# Autodesk Inventor assembly: V2Leg
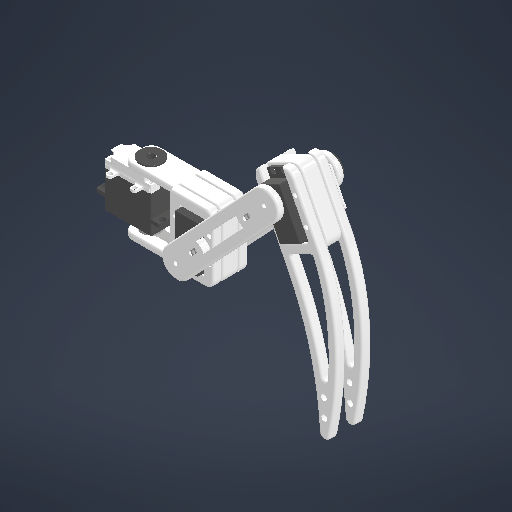
[picture p0: Inventor's stored thumbnail of the model, 512x512]
Saved by Autodesk Inventor 2026.2 (Build 302298010, 298A)
## iProperties
Created: 2026-02-21
Part Number: V2Leg
Document SubType Name: Assembly
Designer: Liam
Author: Liam
## Documents named in this file (12)
- C:\Users\Liam\OneDrive\Documents\Inventor\Hexapod\V2\V2Leg.iam
- C:\Users\Liam\OneDrive\Documents\Inventor\Hexapod\V2\TibiaRight.ipt
- C:\Users\Liam\OneDrive\Documents\Inventor\Hexapod\V2\ServoMount.ipt
- C:\Users\Liam\OneDrive\Documents\Inventor\Hexapod\V2\ServoAssembly.iam
- C:\Users\Liam\OneDrive\Documents\Inventor\Hexapod\V2\TibiaLeft.ipt
- C:\Users\Liam\OneDrive\Documents\Inventor\Hexapod\V2\FemurHornSide.ipt
- C:\Users\Liam\OneDrive\Documents\Inventor\Hexapod\V2\FemurPivotSide.ipt
- C:\Users\Liam\OneDrive\Documents\Inventor\Hexapod\Horn.ipt
- C:\Users\Liam\OneDrive\Documents\Inventor\Hexapod\V2\CoxaHornSide.ipt
- C:\Users\Liam\OneDrive\Documents\Inventor\Hexapod\V2\CoxaPivotSide.ipt
- C:\Users\Liam\OneDrive\Documents\Inventor\Hexapod\V2\CoxaServoCutout.ipt
- C:\Users\Liam\OneDrive\Documents\Inventor\Hexapod\V2\CoxaCableSide.ipt
## Components (15 placed, 11 different names)
1. TibiaRight:1 — Rigid:1
2. ServoMount:1 — Rigid:1, Rigid:2, Rigid:3
3. ServoAssembly:1 [sub-assembly] — Rigid:2, Rotational:5, Rotational:6
4. TibiaLeft:1 — Rigid:3
5. FemurHornSide:1 — Rigid:4, Rigid:9
6. FemurPivotSide:1 — Rotational:5, Rotational:8
7. Horn:1 — Rotational:6, Rigid:4
8. ServoAssembly:2 [sub-assembly] — Rotational:7, Rigid:6, Rotational:8
9. Horn:2 — Rotational:7, Rigid:9
10. CoxaHornSide:1 — Rigid:5, Rigid:6, Rigid:7, Rigid:8, Rigid:10
11. CoxaPivotSide:1 — Rigid:5
12. CoxaServoCutout:1 — Rigid:7
13. CoxaCableSide:1 — Rigid:8
14. ServoAssembly:3 [sub-assembly] — Rotational:9
15. Horn:3 — Rotational:9, Rigid:10
## Relationships (15: WeldJoint 10, RevoluteJoint 5)
- Rigid:1 [WeldJoint]: TibiaRight:1 ↔ ServoMount:1
- Rigid:2 [WeldJoint]: ServoMount:1 ↔ ServoAssembly:1
- Rigid:3 [WeldJoint]: ServoMount:1 ↔ TibiaLeft:1
- Rotational:5 [RevoluteJoint]: ServoAssembly:1 ↔ FemurPivotSide:1
- Rotational:6 [RevoluteJoint]: ServoAssembly:1 ↔ Horn:1
- Rigid:4 [WeldJoint]: FemurHornSide:1 ↔ Horn:1
- Rotational:7 [RevoluteJoint]: ServoAssembly:2 ↔ Horn:2
- Rigid:5 [WeldJoint]: CoxaHornSide:1 ↔ CoxaPivotSide:1
- Rigid:6 [WeldJoint]: ServoAssembly:2 ↔ CoxaHornSide:1
- Rigid:7 [WeldJoint]: CoxaHornSide:1 ↔ CoxaServoCutout:1
- Rigid:8 [WeldJoint]: CoxaHornSide:1 ↔ CoxaCableSide:1
- Rigid:9 [WeldJoint]: FemurHornSide:1 ↔ Horn:2
- Rotational:8 [RevoluteJoint]: FemurPivotSide:1 ↔ ServoAssembly:2
- Rotational:9 [RevoluteJoint]: ServoAssembly:3 ↔ Horn:3
- Rigid:10 [WeldJoint]: CoxaHornSide:1 ↔ Horn:3
